# Autodesk Inventor assembly: tablelegsflange
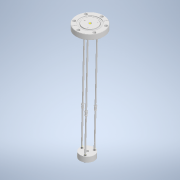
[picture p0: Inventor's stored thumbnail of the model, 180x180]
Saved by Autodesk Inventor 2020 (Build 240168000, 168)
## iProperties
Created: 2019-06-14
Part Number: tablelegsflange
Document SubType Name: Assembly
Designer: ColinP
Author: ColinP
## Documents named in this file (3)
- C:\Users\ColinP\Documents\Inventor\igor\tablelegsflange.iam
- C:\Users\ColinP\Documents\Inventor\igor\updated table+legs.iam
- C:\Users\ColinP\Documents\Inventor\INVENTOR IS_2019June01\FlangeCF275 Blank Modified IS.ipt
## Components (2 placed, 2 different names)
1. updated table+legs:1 [sub-assembly] — Mate:1, Mate:2, Mate:3
2. FlangeCF275 Blank Modified IS:2 — Mate:1, Mate:2, Mate:3
## Relationships (3: Mate 3)
- Mate:1: updated table+legs:1 ↔ FlangeCF275 Blank Modified IS:2
- Mate:2: updated table+legs:1 ↔ FlangeCF275 Blank Modified IS:2
- Mate:3: updated table+legs:1 ↔ FlangeCF275 Blank Modified IS:2
